# Autodesk Inventor assembly: Wheel Assembly
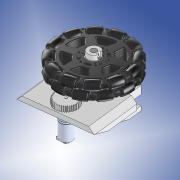
[picture p0: Inventor's stored thumbnail of the model, 180x180]
Saved by Autodesk Inventor 2017 SP1 (Build 210196100, 196)
## iProperties
Created: 2017-08-01
Part Number: Wheel Assembly
Document SubType Name: Assembly
Designer: Zach
Author: Zach
## Documents named in this file (9)
- C:\Users\Zach\Documents\GitHub\cr-laundry-robot\src\Base 2\Wheel Assembly\Wheel Assembly.iam
- C:\Users\Zach\Documents\GitHub\cr-laundry-robot\src\Base 2\Wheel Assembly\WA001.ipt
- C:\Users\Zach\Documents\GitHub\cr-laundry-robot\lib\Omni Wheel 6in\217-2585.ipt
- C:\Users\Zach\Documents\GitHub\cr-laundry-robot\lib\28x12x8mm Bearing.ipt
- C:\Users\Zach\Documents\GitHub\cr-laundry-robot\src\Base 2\Wheel Assembly\WA003.ip.ipt
- C:\Users\Zach\Documents\GitHub\cr-laundry-robot\src\Base 2\Wheel Assembly\WA004.ipt
- C:\Users\Zach\Documents\GitHub\cr-laundry-robot\lib\DC Motor with Encoder\Motor.ipt
- C:\Users\Zach\Documents\GitHub\cr-laundry-robot\src\Base 2\Wheel Assembly\Wheel Assembly\Design Accelerator\Spur Gears1.iam
- C:\Users\Zach\Documents\GitHub\cr-laundry-robot\src\Base 2\Wheel Assembly\WA002.ipt
## Components (12 placed, 8 different names)
1. WA001:1 — Mate:3, Mate:7, Mate:9, Mate:10, Mate:11, Mate:21, Mate:23, Mate:29, Mate:30, Mate:31
2. 217-2585:1 — Mate:1, Flush:1, Mate:2, Flush:2, Mate:8, Mate:27, Mate:28
3. 28x12x8mm Bearing:1 — Mate:1, Flush:1, Mate:3, Mate:32
4. 28x12x8mm Bearing:2 — Mate:2, Flush:2
5. WA003.ip:1 — Mate:7, Mate:8, Mate:29
6. WA004:1 — Mate:9, Mate:14, Mate:15, Mate:16, Mate:17, Mate:18, Mate:19, Mate:20, Mate:24, Mate:26
7. Motor:1 — Mate:14, Mate:15, Mate:16, Mate:25
8. 28x12x8mm Bearing:3 — Mate:19, Mate:20
9. 28x12x8mm Bearing:4 — Mate:17, Mate:18
10. WA003.ip:2 — Mate:21, Mate:30
11. Spur Gears:1 [sub-assembly] — Mate:23, Mate:24, Mate:25, Mate:26, Mate:27, Mate:28
12. WA002:1 — Mate:31, Mate:32
## Relationships (28: Mate 26, Flush 2)
- Mate:1: 217-2585:1 ↔ 28x12x8mm Bearing:1
- Flush:1: 217-2585:1 ↔ 28x12x8mm Bearing:1
- Mate:2: 217-2585:1 ↔ 28x12x8mm Bearing:2
- Flush:2: 217-2585:1 ↔ 28x12x8mm Bearing:2
- Mate:3: WA001:1 ↔ 28x12x8mm Bearing:1
- Mate:7: WA001:1 ↔ WA003.ip:1
- Mate:8: 217-2585:1 ↔ WA003.ip:1
- Mate:9: WA001:1 ↔ WA004:1
- Mate:10: WA001:1
- Mate:11: WA001:1
- Mate:14: WA004:1 ↔ Motor:1
- Mate:15: WA004:1 ↔ Motor:1
- Mate:16: WA004:1 ↔ Motor:1
- Mate:17: WA004:1 ↔ 28x12x8mm Bearing:4
- Mate:18: WA004:1 ↔ 28x12x8mm Bearing:4
- Mate:19: WA004:1 ↔ 28x12x8mm Bearing:3
- Mate:20: WA004:1 ↔ 28x12x8mm Bearing:3
- Mate:21: WA001:1 ↔ WA003.ip:2
- Mate:23: WA001:1 ↔ Spur Gears:1
- Mate:24: WA004:1 ↔ Spur Gears:1
- Mate:25: Motor:1 ↔ Spur Gears:1
- Mate:26: WA004:1 ↔ Spur Gears:1
- Mate:27: 217-2585:1 ↔ Spur Gears:1
- Mate:28: 217-2585:1 ↔ Spur Gears:1
- Mate:29: WA001:1 ↔ WA003.ip:1
- Mate:30: WA001:1 ↔ WA003.ip:2
- Mate:31: WA001:1 ↔ WA002:1
- Mate:32: 28x12x8mm Bearing:1 ↔ WA002:1
